# Autodesk Inventor assembly: ЛЦМК.30000,00,00,00 СБ Шлем
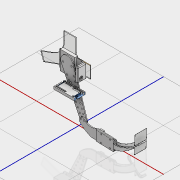
[picture p0: Inventor's stored thumbnail of the model, 180x180]
Saved by Autodesk Inventor 2021.2 (Build 252289000, 289)
## iProperties
Created: 2025-11-22
Part Number: ЛЦМК.30000,00,00,00 СБ Шлем
Document SubType Name: Assembly
Designer: Захаров
Author: Захаров
## Documents named in this file (6)
- C:\Users\User\Documents\CaseARHead1\ЛЦМК.30000.00.00.00 СБ Шлем.iam
- ЛЦМК.30000.00.00.00 СБ Шлем.iam
- C:\Users\User\Documents\CaseARHead1\ЛЦМК.30000.10.00.00 Корпус XIAO\ЛЦМК.30000.10.00.00 СБ Корпус XIAO.iam
- C:\Users\User\Documents\CaseARHead1\ЛЦМК.30000.20.00.00 Держатель OLED\ЛЦМК.30000.20.00.00 СБ Держатель OLED.iam
- C:\Users\User\Documents\CaseARHead1\ЛЦМК.30000.30.00.00 Крепление\ЛЦМК.30000.30.00.00 СБ Крепление.iam
- C:\Users\User\Documents\CaseARHead1\Заготовки\ЛЦМК.30000.10.00.01 Основание.ipt
## Components (4 placed, 4 different names)
1. ЛЦМК.30000.10.00.00 СБ Корпус XIAO:1 [sub-assembly]
2. ЛЦМК.30000.20.00.00 СБ Держатель OLED:1 [sub-assembly] — Вставка:1, Угол:1
3. ЛЦМК.30000.30.00.00 СБ Крепление:1 [sub-assembly] — Вставка:1, Угол:1, Совмещение:1
4. ЛЦМК.30000.10.00.01 Основание:1 — Совмещение:1
## Relationships (3: Insert 1, Angle 1, Mate 1)
- Вставка:1 [Insert]: ЛЦМК.30000.20.00.00 СБ Держатель OLED:1 ↔ ЛЦМК.30000.30.00.00 СБ Крепление:1
- Угол:1 [Angle] (70 deg): ЛЦМК.30000.20.00.00 СБ Держатель OLED:1 ↔ ЛЦМК.30000.30.00.00 СБ Крепление:1
- Совмещение:1 [Mate]: ЛЦМК.30000.30.00.00 СБ Крепление:1 ↔ ЛЦМК.30000.10.00.01 Основание:1
